# Autodesk Inventor assembly: NP18-12
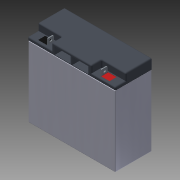
[picture p0: Inventor's stored thumbnail of the model, 180x180]
Saved by Autodesk Inventor 2013 (Build 170138000, 138)
## iProperties
Category: Electrical
Company: Autodesk Inc.
Created: 2011-12-13
Part Number: NP18-12
Document SubType Name: Assembly
Designer: Autodesk
Description: Battery, ,12 volt, 18 AH, Non-spillable
Mass: 6259.58 g
Surface Area: 1482.32 cm^2
Volume: 2177.92 cm^3
Author: Autodesk Inc.
## Documents named in this file (3)
- C:\Users\Arpan\Documents\GitHub\frc2013CAD\Electrical\ELEC_Battery_NP18-12B.iam
- C:\Users\Arpan\Documents\GitHub\frc2013CAD\Electrical\Electrical_Yuasa_NP18-12_Top.ipt
- C:\Users\Arpan\Documents\GitHub\frc2013CAD\Electrical\Electrical_Yuasa_Np18-12_Middle.ipt
## Components (2 placed, 2 different names)
1. Electrical_Yuasa_NP18-12_Top:1 — Flush:1
2. Electrical_Yuasa_Np18-12_Middle:1 — Flush:1
## Relationships (1: Flush 1)
- Flush:1: Electrical_Yuasa_NP18-12_Top:1 ↔ Electrical_Yuasa_Np18-12_Middle:1
